# Autodesk Inventor assembly: Assembly2
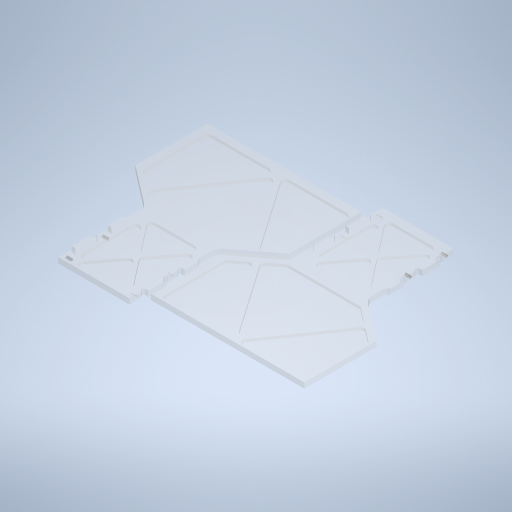
[picture p0: Inventor's stored thumbnail of the model, 512x512]
Saved by Autodesk Inventor 2024 (Build 280153000, 153)
## iProperties
Created: 2023-12-22
Part Number: Assembly2
Document SubType Name: Assembly
Designer: right
Author: right
## Documents named in this file (2)
- C:\Users\right\OneDrive\ドキュメント\Inventor\V2二足Light＿仮\Assembly2.iam
- C:\Users\right\OneDrive\ドキュメント\Inventor\V2二足Light＿仮\new_hera.ipt
## Components (2 placed, 1 different names)
1. new_hera:1 — メイト:1, メイト:2, フラッシュ:1
2. new_hera:2 — メイト:1, メイト:2, フラッシュ:1
## Relationships (3: Mate 2, Flush 1)
- メイト:1 [Mate] (2.2 mm): new_hera:1 ↔ new_hera:2
- メイト:2 [Mate] (2.2 mm): new_hera:1 ↔ new_hera:2
- フラッシュ:1 [Flush]: new_hera:1 ↔ new_hera:2
